# Autodesk Inventor assembly: Intake Angled
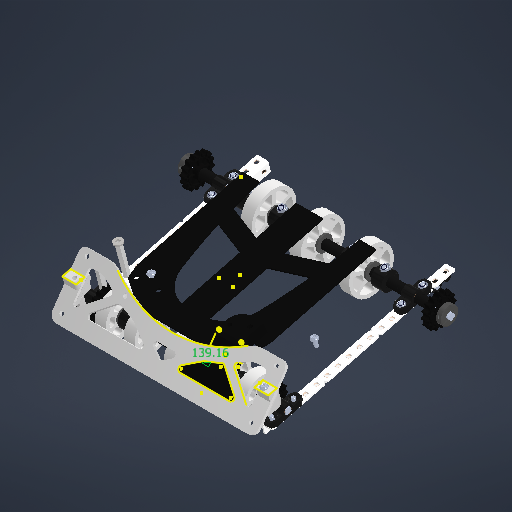
[picture p0: Inventor's stored thumbnail of the model, 512x512]
Saved by Autodesk Inventor 2025 (Build 290162000, 162)
## iProperties
Created: 2024-12-18
Part Number: Intake Angled
Document SubType Name: Assembly
Designer: Juan
Author: Juan
## Documents named in this file (38)
- C:\Users\Juan\Documents\GitHub\ATUM-VRC-High-Stakes-CAD\Robot\Subassemblies\Intake Angled.iam
- C:\Users\Juan\Documents\GitHub\ATUM-VRC-High-Stakes-CAD\VEX-CAD-Inventor\Motion\Shaft HS\Shaft HS\Shaft HS 9.0 in.ipt
- C:\Users\Juan\Documents\GitHub\ATUM-VRC-High-Stakes-CAD\VEX-CAD-Inventor\Motion\Shaft HS\Shaft HS.ipt
- C:\Users\Juan\Documents\GitHub\ATUM-VRC-High-Stakes-CAD\VEX-CAD-Inventor\Structure\Angle\Aluminum 1x1\Alu Angle 1x1x17.ipt
- C:\Users\Juan\Documents\GitHub\ATUM-VRC-High-Stakes-CAD\VEX-CAD-Inventor\Motion\Shaft HS\HS Pillow Bearing Block.ipt
- C:\Users\Juan\Documents\GitHub\ATUM-VRC-High-Stakes-CAD\VEX-CAD-Inventor\Motion\Sprockets\6P Sprocket\6P 16T Sprocket, No Insert.iam
- C:\Users\Juan\Documents\GitHub\ATUM-VRC-High-Stakes-CAD\VEX-CAD-Inventor\Motion\Sprockets\6P Sprocket.iam
- C:\Users\Juan\Documents\GitHub\ATUM-VRC-High-Stakes-CAD\VEX-CAD-Inventor\Structure\Hardware\Screw Steel - Star\SScrew Star Threaded .375.ipt
- C:\Users\Juan\Documents\GitHub\ATUM-VRC-High-Stakes-CAD\VEX-CAD-Inventor\Structure\Hardware\Screw Steel - Star.ipt
- C:\Users\Juan\Documents\GitHub\ATUM-VRC-High-Stakes-CAD\VEX-CAD-Inventor\Structure\Standoff\Standoff 1.50.ipt
- C:\Users\Juan\Documents\GitHub\ATUM-VRC-High-Stakes-CAD\VEX-CAD-Inventor\Structure\Standoff.ipt
- C:\Users\Juan\Documents\GitHub\ATUM-VRC-High-Stakes-CAD\VEX-CAD-Inventor\Motion\1-Post Bearing Flat Hex Retainer.ipt
- C:\Users\Juan\Documents\GitHub\ATUM-VRC-High-Stakes-CAD\VEX-CAD-Inventor\Motion\Shaft HS\Shaft HS\Shaft HS 12.0 in.ipt
- C:\Users\Juan\Documents\GitHub\ATUM-VRC-High-Stakes-CAD\VEX-CAD-Inventor\Motion\Shaft HS\HS Shaft Collar.ipt
- C:\Users\Juan\Documents\GitHub\ATUM-VRC-High-Stakes-CAD\VEX-CAD-Inventor\Motion\Shaft HS\HS Spacer\HSpacer .5000.ipt
- C:\Users\Juan\Documents\GitHub\ATUM-VRC-High-Stakes-CAD\VEX-CAD-Inventor\Motion\Shaft HS\HS Spacer.ipt
- C:\Users\Juan\Documents\GitHub\ATUM-VRC-High-Stakes-CAD\VEX-CAD-Inventor\Motion\Shaft HS\Low Profile HS Shaft Collar.ipt
- C:\Users\Juan\Documents\GitHub\ATUM-VRC-High-Stakes-CAD\VEX-CAD-Inventor\Motion\Shaft HS\HS Spacer\HSpacer .2500.ipt
- C:\Users\Juan\Documents\GitHub\ATUM-VRC-High-Stakes-CAD\Robot\Subassemblies\2.0 Flex Wheel with Insert.iam
- C:\Users\Juan\Documents\GitHub\ATUM-VRC-High-Stakes-CAD\VEX-CAD-Inventor\Structure\Hardware\Nut Thin Nylock.ipt
- C:\Users\Juan\Documents\GitHub\ATUM-VRC-High-Stakes-CAD\VEX-CAD-Inventor\Structure\Hardware\Screw Steel - Star\SScrew Star Smooth .625.ipt
- C:\Users\Juan\Documents\GitHub\ATUM-VRC-High-Stakes-CAD\VEX-CAD-Inventor\Motion\Shaft HS\HS Spacer\HSpacer .1250.ipt
- C:\Users\Juan\Documents\GitHub\ATUM-VRC-High-Stakes-CAD\VEX-CAD-Inventor\Motion\Shaft HS\HS Spacer\HSpacer .0625.ipt
- C:\Users\Juan\Documents\GitHub\ATUM-VRC-High-Stakes-CAD\VEX-CAD-Inventor\Structure\Hardware\Screw Steel - Star\SScrew Star Smooth .375.ipt
- C:\Users\Juan\Documents\GitHub\ATUM-VRC-High-Stakes-CAD\Robot\Subassemblies\1.625 Flex Wheel with Insert.iam
- C:\Users\Juan\Documents\GitHub\ATUM-VRC-High-Stakes-CAD\Protobot\Intake (Metal).ipt
- C:\Users\Juan\Documents\GitHub\ATUM-VRC-High-Stakes-CAD\VEX-CAD-Inventor\Motion\Spacers\Washer Steel\SWasher .375 OD x .062500.ipt
- C:\Users\Juan\Documents\GitHub\ATUM-VRC-High-Stakes-CAD\VEX-CAD-Inventor\Motion\Spacers\Washer Steel.ipt
- C:\Users\Juan\Documents\GitHub\ATUM-VRC-High-Stakes-CAD\VEX-CAD-Inventor\Motion\Spacers\Washer Steel\SWasher .375 OD x .015625.ipt
- C:\Users\Juan\Documents\GitHub\ATUM-VRC-High-Stakes-CAD\Protobot\Intake Hood.ipt
- C:\Users\Juan\Documents\GitHub\ATUM-VRC-High-Stakes-CAD\VEX-CAD-Inventor\Structure\Standoff\Standoff .75.ipt
- C:\Users\Juan\Documents\GitHub\ATUM-VRC-High-Stakes-CAD\VEX-CAD-Inventor\Motion\Spacers\Spacer Nylon .375 OD\NSpacer .375 OD x .500.ipt
- C:\Users\Juan\Documents\GitHub\ATUM-VRC-High-Stakes-CAD\VEX-CAD-Inventor\Motion\Spacers\Spacer Nylon .375 OD.ipt
- C:\Users\Juan\Documents\GitHub\ATUM-VRC-High-Stakes-CAD\Protobot\Intake Angle Mount.ipt
- C:\Users\Juan\Documents\GitHub\ATUM-VRC-High-Stakes-CAD\Protobot\Intake Angle Mount_MIR.ipt
- C:\Users\Juan\Documents\GitHub\ATUM-VRC-High-Stakes-CAD\Protobot\Intake Angle Spacer.ipt
- C:\Users\Juan\Documents\GitHub\ATUM-VRC-High-Stakes-CAD\Protobot\Intake Angle Spacer_MIR.ipt
- C:\Users\Juan\Documents\GitHub\ATUM-VRC-High-Stakes-CAD\Protobot\Intake Hood Mount.ipt
## Components (103 placed, 30 different names)
1. Shaft HS 9.0 in:1
2. Alu Angle 1x1x17:1
3. HS Pillow Bearing Block:4
4. Alu Angle 1x1x17:2 — Rigid:32, Rigid:56
5. HS Pillow Bearing Block:1 — Rigid:57
6. HS Pillow Bearing Block:2 — Rotational:1
7. 6P 16T Sprocket, No Insert:1 [sub-assembly]
8. 6P 16T Sprocket, No Insert:2 [sub-assembly]
9. SScrew Star Threaded .375:1
10. Standoff 1.50:2
11. Standoff 1.50:3
12. 1-Post Bearing Flat Hex Retainer:1
13. HS Pillow Bearing Block:3
14. Shaft HS 12.0 in:2
15. 6P 16T Sprocket, No Insert:3 [sub-assembly]
16. 6P 16T Sprocket, No Insert:4 [sub-assembly]
17. HS Shaft Collar:1
18. HS Shaft Collar:2
19. HSpacer .5000:1
20. HSpacer .5000:2
21. HSpacer .5000:3
22. HSpacer .5000:4
23. Low Profile HS Shaft Collar:1
24. Low Profile HS Shaft Collar:2
25. HS Shaft Collar:3
26. HS Shaft Collar:4
27. HSpacer .2500:5
28. HSpacer .2500:6
29. 2.0 Flex Wheel with Insert:1 [sub-assembly]
30. 1-Post Bearing Flat Hex Retainer:2
31. 2.0 Flex Wheel with Insert:2 [sub-assembly]
32. 2.0 Flex Wheel with Insert:3 [sub-assembly]
33. HSpacer .5000:7
34. Nut Thin Nylock:1
35. HSpacer .5000:8
36. SScrew Star Smooth .625:2
37. SScrew Star Smooth .625:3
38. SScrew Star Smooth .625:4
39. SScrew Star Smooth .625:5
40. Nut Thin Nylock:2
41. Nut Thin Nylock:3
42. Nut Thin Nylock:4
43. HSpacer .5000:9
44. HSpacer .5000:10
45. HSpacer .1250:11
46. HSpacer .1250:12
47. HSpacer .0625:13
48. HSpacer .1250:14
49. HSpacer .1250:15
50. HSpacer .0625:16
51. HSpacer .0625:17
52. Nut Thin Nylock:5
53. Nut Thin Nylock:6
54. Nut Thin Nylock:7
55. Nut Thin Nylock:8
56. SScrew Star Smooth .375:6
57. SScrew Star Smooth .375:7
58. SScrew Star Smooth .375:8
59. SScrew Star Smooth .375:9
60. SScrew Star Smooth .375:14
61. SScrew Star Smooth .375:15
62. SScrew Star Smooth .375:16
63. SScrew Star Smooth .375:17
64. 1.625 Flex Wheel with Insert:1 [sub-assembly]
65. 1.625 Flex Wheel with Insert:2 [sub-assembly]
66. 1.625 Flex Wheel with Insert:3 [sub-assembly]
67. 1.625 Flex Wheel with Insert:4 [sub-assembly]
68. 1.625 Flex Wheel with Insert:5 [sub-assembly]
69. HSpacer .5000:18
70. HSpacer .1250:19
71. HSpacer .1250:20
72. HSpacer .5000:21
73. HSpacer .5000:22
74. HSpacer .5000:23
75. HS Shaft Collar:5
76. Nut Thin Nylock:9
77. SScrew Star Smooth .625:18
78. HS Shaft Collar:6
79. Nut Thin Nylock:10
80. SScrew Star Smooth .625:19
81. HSpacer .1250:24
82. HSpacer .1250:25
83. Standoff 1.50:5 — Rigid:32, Rigid:36
84. SWasher .375 OD x .062500:5 — Rigid:36
85. SWasher .375 OD x .015625:6
86. Intake Hood:1 — Rigid:50, Mate:127
87. SScrew Star Smooth .375:29 — Mate:127
88. SScrew Star Smooth .375:32
89. Nut Thin Nylock:12 — Rigid:50
90. Nut Thin Nylock:17
91. SScrew Star Smooth .375:33 — Rigid:56
92. Standoff .75:7 — Rotational:1, Mate:132, Mate:133
93. Standoff .75:8 — Rigid:57, Rigid:58, Mate:130
94. Intake (Metal):1
95. NSpacer .375 OD x .500:1 — Rigid:58, Mate:128
96. Intake (Metal):2 — Flush:2, Mate:129, Flush:3, Mate:131, Mate:134, Mate:135, Mate:137, Flush:4, Mate:139, Mate:140, Mate:141
97. Intake Angle Mount:1 — Mate:128, Flush:2, Mate:129, Mate:130, Mate:136
98. Intake Angle Mount_MIR:1 — Flush:3, Mate:131, Mate:132, Mate:133, Mate:134, Mate:138
99. Intake Angle Spacer:1 — Mate:135, Mate:136, Rigid:59
100. Intake Angle Spacer_MIR:1 — Mate:137, Mate:138, Flush:4
101. SScrew Star Smooth .375:34 — Rigid:59
102. Intake Hood Mount:1 — Mate:139, Mate:140, Mate:141
103. SScrew Star Smooth .375:35
## Relationships (175: Mate 126, WeldJoint 34, CylindricalJoint 9, Flush 4, Angle 1, RevoluteJoint 1)
- [Mate]: Alu Angle 1x1x17:1 ↔ HS Pillow Bearing Block:1
- [Mate]: Alu Angle 1x1x17:1 ↔ HS Pillow Bearing Block:1
- [Mate]: Alu Angle 1x1x17:1 ↔ HS Pillow Bearing Block:1
- [Mate]: Shaft HS 9.0 in:1 ↔ HS Pillow Bearing Block:1
- [Mate]: Alu Angle 1x1x17:2 ↔ HS Pillow Bearing Block:2
- [Mate]: Alu Angle 1x1x17:2 ↔ HS Pillow Bearing Block:2
- [Mate]: Alu Angle 1x1x17:2 ↔ HS Pillow Bearing Block:2
- [Mate]: Shaft HS 9.0 in:1 ↔ HS Pillow Bearing Block:2
- [Mate]: Shaft HS 9.0 in:1 ↔ 6P 16T Sprocket, No Insert:2
- [Mate]: Shaft HS 9.0 in:1 ↔ 6P 16T Sprocket, No Insert:1
- [Mate]: Alu Angle 1x1x17:1 ↔ SScrew Star Threaded .375:1
- [Mate]: Alu Angle 1x1x17:1 ↔ 6P 16T Sprocket, No Insert:2
- [Mate]: Alu Angle 1x1x17:1 ↔ SScrew Star Threaded .375:1
- [Mate]: Alu Angle 1x1x17:1 ↔ Alu Angle 1x1x17:2
- [Mate]: HS Pillow Bearing Block:1 ↔ Standoff 1.50:2
- [Mate]: HS Pillow Bearing Block:1 ↔ Standoff 1.50:2
- [Mate]: HS Pillow Bearing Block:2 ↔ Standoff 1.50:3
- [Mate]: HS Pillow Bearing Block:2 ↔ Standoff 1.50:3
- [Mate]: Alu Angle 1x1x17:2 ↔ HS Pillow Bearing Block:3
- [Mate]: Alu Angle 1x1x17:2 ↔ HS Pillow Bearing Block:3
- [Mate]: Alu Angle 1x1x17:2 ↔ HS Pillow Bearing Block:3
- [Mate]: Shaft HS 12.0 in:2 ↔ 6P 16T Sprocket, No Insert:3
- [Mate]: Shaft HS 12.0 in:2 ↔ 6P 16T Sprocket, No Insert:4
- [Mate]: Shaft HS 12.0 in:2 ↔ 2.0 Flex Wheel with Insert:3
- [Mate]: Shaft HS 12.0 in:2 ↔ 2.0 Flex Wheel with Insert:2
- [Mate]: Shaft HS 12.0 in:2 ↔ 2.0 Flex Wheel with Insert:1
- [Mate]: Shaft HS 12.0 in:2 ↔ HSpacer .5000:4
- [Mate]: Shaft HS 12.0 in:2 ↔ HSpacer .5000:4
- [Mate]: Shaft HS 12.0 in:2 ↔ HS Shaft Collar:1
- [Mate]: Shaft HS 12.0 in:2 ↔ HS Shaft Collar:1
- [Mate]: Shaft HS 12.0 in:2 ↔ HSpacer .5000:1
- [Mate]: Shaft HS 12.0 in:2 ↔ HSpacer .5000:1
- [Mate]: HSpacer .5000:1 ↔ HSpacer .5000:4
- [Mate]: HS Shaft Collar:1 ↔ HSpacer .5000:4
- [Mate]: HS Shaft Collar:1 ↔ 2.0 Flex Wheel with Insert:3
- [Mate]: HSpacer .5000:1 ↔ 2.0 Flex Wheel with Insert:2
- [Mate]: Shaft HS 12.0 in:2 ↔ HS Shaft Collar:2
- [Mate]: Shaft HS 12.0 in:2 ↔ HS Shaft Collar:2
- [Mate]: Shaft HS 12.0 in:2 ↔ HSpacer .5000:3
- [Mate]: Shaft HS 12.0 in:2 ↔ HSpacer .5000:3
- [Mate]: Shaft HS 12.0 in:2 ↔ HSpacer .5000:2
- [Mate]: Shaft HS 12.0 in:2 ↔ HSpacer .5000:2
- [Mate]: HSpacer .5000:2 ↔ 2.0 Flex Wheel with Insert:2
- [Mate]: HSpacer .5000:2 ↔ HSpacer .5000:3
- [Mate]: HS Shaft Collar:2 ↔ HSpacer .5000:3
- [Mate]: HS Shaft Collar:2 ↔ 2.0 Flex Wheel with Insert:1
- [Mate] (36.1696 mm): Alu Angle 1x1x17:1 ↔ 2.0 Flex Wheel with Insert:3
- [Mate]: Shaft HS 12.0 in:2 ↔ Low Profile HS Shaft Collar:2
- [Mate]: Shaft HS 12.0 in:2 ↔ Low Profile HS Shaft Collar:2
- [Mate]: 6P 16T Sprocket, No Insert:3 ↔ Low Profile HS Shaft Collar:2
- [Mate]: Shaft HS 12.0 in:2 ↔ Low Profile HS Shaft Collar:1
- [Mate]: Shaft HS 12.0 in:2 ↔ Low Profile HS Shaft Collar:1
- [Mate]: 6P 16T Sprocket, No Insert:4 ↔ Low Profile HS Shaft Collar:1
- [Mate]: Shaft HS 12.0 in:2 ↔ HS Shaft Collar:3
- [Mate]: Shaft HS 12.0 in:2 ↔ HS Shaft Collar:3
- [Mate]: Shaft HS 12.0 in:2 ↔ HS Shaft Collar:4
- [Mate]: Shaft HS 12.0 in:2 ↔ HS Shaft Collar:4
- [Mate]: Shaft HS 12.0 in:2 ↔ HSpacer .2500:5
- [Mate]: Shaft HS 12.0 in:2 ↔ HSpacer .2500:5
- [Mate]: Shaft HS 12.0 in:2 ↔ HSpacer .2500:6
- [Mate]: Shaft HS 12.0 in:2 ↔ HSpacer .2500:6
- [Mate]: HSpacer .2500:6 ↔ 2.0 Flex Wheel with Insert:3
- [Mate]: HSpacer .2500:5 ↔ 2.0 Flex Wheel with Insert:1
- [Mate]: HS Shaft Collar:4 ↔ HSpacer .2500:5
- [Mate]: HS Shaft Collar:3 ↔ HSpacer .2500:6
- [WeldJoint]: HS Shaft Collar:3 ↔ SScrew Star Smooth .625:2
- [WeldJoint]: HS Shaft Collar:1 ↔ SScrew Star Smooth .625:5
- [WeldJoint]: HS Shaft Collar:2 ↔ SScrew Star Smooth .625:4
- [WeldJoint]: HS Shaft Collar:4 ↔ SScrew Star Smooth .625:3
- [WeldJoint]: HS Shaft Collar:3 ↔ Nut Thin Nylock:1
- [WeldJoint]: HS Shaft Collar:4 ↔ Nut Thin Nylock:2
- [WeldJoint]: HS Shaft Collar:2 ↔ Nut Thin Nylock:3
- [WeldJoint]: HS Shaft Collar:1 ↔ Nut Thin Nylock:4
- [WeldJoint]: HS Shaft Collar:3 ↔ HSpacer .5000:7
- [WeldJoint]: HS Shaft Collar:4 ↔ HSpacer .5000:9
- [Mate]: Shaft HS 12.0 in:2 ↔ HSpacer .5000:8
- [Mate]: 6P 16T Sprocket, No Insert:3 ↔ HSpacer .5000:8
- [Mate]: Shaft HS 12.0 in:2 ↔ HSpacer .5000:10
- [Mate]: 6P 16T Sprocket, No Insert:4 ↔ HSpacer .5000:10
- [Mate]: Shaft HS 12.0 in:2 ↔ HSpacer .1250:12
- [Mate]: HSpacer .5000:10 ↔ HSpacer .1250:12
- [Mate]: HSpacer .5000:9 ↔ HSpacer .1250:11
- [Mate]: HSpacer .5000:9 ↔ HSpacer .1250:11
- [Mate]: HSpacer .1250:11 ↔ HSpacer .0625:13
- [Mate]: HSpacer .1250:11 ↔ HSpacer .0625:13
- [Mate]: HSpacer .5000:8 ↔ HSpacer .1250:14
- [Mate]: HSpacer .5000:8 ↔ HSpacer .1250:14
- [Mate]: HSpacer .1250:14 ↔ HSpacer .0625:16
- [Mate]: HSpacer .1250:14 ↔ HSpacer .0625:16
- [Mate]: HSpacer .5000:7 ↔ HSpacer .1250:15
- [Mate]: HSpacer .5000:7 ↔ HSpacer .1250:15
- [Mate]: HSpacer .1250:15 ↔ HSpacer .0625:17
- [Mate]: HSpacer .1250:15 ↔ HSpacer .0625:17
- [WeldJoint]: HS Pillow Bearing Block:3 ↔ Nut Thin Nylock:7
- [WeldJoint]: HS Pillow Bearing Block:3 ↔ Nut Thin Nylock:8
- [WeldJoint]: Alu Angle 1x1x17:1 ↔ SScrew Star Smooth .375:6
- [WeldJoint]: Alu Angle 1x1x17:1 ↔ SScrew Star Smooth .375:7
- [WeldJoint]: Alu Angle 1x1x17:2 ↔ SScrew Star Smooth .375:9
- [WeldJoint]: Alu Angle 1x1x17:2 ↔ SScrew Star Smooth .375:8
- [WeldJoint]: Alu Angle 1x1x17:2 ↔ SScrew Star Smooth .375:15
- [WeldJoint]: Alu Angle 1x1x17:2 ↔ SScrew Star Smooth .375:14
- [WeldJoint]: Alu Angle 1x1x17:1 ↔ SScrew Star Smooth .375:17
- [WeldJoint]: Alu Angle 1x1x17:1 ↔ SScrew Star Smooth .375:16
- [CylindricalJoint]: Shaft HS 9.0 in:1 ↔ 1.625 Flex Wheel with Insert:1
- [CylindricalJoint]: Shaft HS 9.0 in:1 ↔ 1.625 Flex Wheel with Insert:5
- [Mate]: 1.625 Flex Wheel with Insert:5 ↔ HSpacer .5000:18
- [Mate]: 1.625 Flex Wheel with Insert:5 ↔ HSpacer .1250:19
- [Mate]: 1.625 Flex Wheel with Insert:5 ↔ HSpacer .1250:19
- [Mate]: HSpacer .5000:18 ↔ HSpacer .1250:19
- [Mate]: 1.625 Flex Wheel with Insert:5 ↔ HSpacer .1250:20
- [Mate]: 1.625 Flex Wheel with Insert:5 ↔ HSpacer .1250:20
- [Mate]: 1.625 Flex Wheel with Insert:5 ↔ HSpacer .5000:21
- [Mate]: HSpacer .1250:20 ↔ HSpacer .5000:21
- [Mate]: 1.625 Flex Wheel with Insert:5 ↔ HSpacer .5000:23
- [Mate]: HSpacer .5000:18 ↔ HSpacer .5000:23
- [Mate]: 1.625 Flex Wheel with Insert:5 ↔ HSpacer .5000:22
- [Mate]: HSpacer .5000:21 ↔ HSpacer .5000:22
- [Mate]: 1.625 Flex Wheel with Insert:1 ↔ HSpacer .5000:23
- [CylindricalJoint]: Shaft HS 9.0 in:1 ↔ 1.625 Flex Wheel with Insert:4
- [Mate]: 1.625 Flex Wheel with Insert:4 ↔ HSpacer .5000:22
- [CylindricalJoint]: Shaft HS 9.0 in:1 ↔ 1.625 Flex Wheel with Insert:3
- [CylindricalJoint]: Shaft HS 9.0 in:1 ↔ 1.625 Flex Wheel with Insert:2
- [WeldJoint]: HS Shaft Collar:5 ↔ SScrew Star Smooth .625:18
- [WeldJoint]: HS Shaft Collar:5 ↔ Nut Thin Nylock:9
- [WeldJoint]: HS Shaft Collar:6 ↔ SScrew Star Smooth .625:19
- [WeldJoint]: HS Shaft Collar:6 ↔ Nut Thin Nylock:10
- [CylindricalJoint]: Shaft HS 9.0 in:1 ↔ HS Shaft Collar:5
- [CylindricalJoint]: Shaft HS 9.0 in:1 ↔ HS Shaft Collar:6
- [Mate]: 6P 16T Sprocket, No Insert:1 ↔ 1.625 Flex Wheel with Insert:2
- [Mate]: 1.625 Flex Wheel with Insert:2 ↔ HS Shaft Collar:6
- [Mate]: 6P 16T Sprocket, No Insert:2 ↔ 1.625 Flex Wheel with Insert:3
- [Mate]: 1.625 Flex Wheel with Insert:3 ↔ HS Shaft Collar:5
- [Mate]: Alu Angle 1x1x17:2 ↔ 6P 16T Sprocket, No Insert:1
- [Flush]: HS Shaft Collar:5 ↔ HS Shaft Collar:6
- [Angle] (0 deg): Shaft HS 9.0 in:1 ↔ HS Shaft Collar:5
- [CylindricalJoint]: Shaft HS 9.0 in:1 ↔ HSpacer .1250:25
- [Mate]: HS Shaft Collar:5 ↔ HSpacer .1250:25
- [Mate]: 1.625 Flex Wheel with Insert:1 ↔ HSpacer .1250:25
- [CylindricalJoint]: Shaft HS 9.0 in:1 ↔ HSpacer .1250:24
- [Mate]: 1.625 Flex Wheel with Insert:4 ↔ HSpacer .1250:24
- [Mate]: Alu Angle 1x1x17:1 ↔ HS Pillow Bearing Block:4
- [Mate]: Alu Angle 1x1x17:1 ↔ HS Pillow Bearing Block:4
- [Mate]: Alu Angle 1x1x17:1 ↔ HS Pillow Bearing Block:4
- [Mate]: HS Pillow Bearing Block:4 ↔ Shaft HS 12.0 in:2
- [WeldJoint]: HS Pillow Bearing Block:4 ↔ Nut Thin Nylock:6
- [WeldJoint]: HS Pillow Bearing Block:4 ↔ Nut Thin Nylock:5
- [Mate]: Alu Angle 1x1x17:1 ↔ 1-Post Bearing Flat Hex Retainer:2
- [Mate]: SScrew Star Threaded .375:1 ↔ 1-Post Bearing Flat Hex Retainer:2
- Rigid:32 [WeldJoint]: Alu Angle 1x1x17:2 ↔ Standoff 1.50:5
- [WeldJoint]: SWasher .375 OD x .062500:5 ↔ SWasher .375 OD x .015625:6
- Rigid:36 [WeldJoint]: Standoff 1.50:5 ↔ SWasher .375 OD x .062500:5
- Rigid:50 [WeldJoint]: Intake Hood:1 ↔ Nut Thin Nylock:12
- Rigid:56 [WeldJoint]: Alu Angle 1x1x17:2 ↔ SScrew Star Smooth .375:33
- Mate:127: Intake Hood:1 ↔ SScrew Star Smooth .375:29
- Rigid:57 [WeldJoint]: HS Pillow Bearing Block:1 ↔ Standoff .75:8
- Rotational:1 [RevoluteJoint]: HS Pillow Bearing Block:2 ↔ Standoff .75:7
- Rigid:58 [WeldJoint]: Standoff .75:8 ↔ NSpacer .375 OD x .500:1
- Mate:128: NSpacer .375 OD x .500:1 ↔ Intake Angle Mount:1
- Flush:2: Intake (Metal):2 ↔ Intake Angle Mount:1
- Mate:129: Intake (Metal):2 ↔ Intake Angle Mount:1
- Mate:130: Standoff .75:8 ↔ Intake Angle Mount:1
- Flush:3: Intake (Metal):2 ↔ Intake Angle Mount_MIR:1
- Mate:131: Intake (Metal):2 ↔ Intake Angle Mount_MIR:1
- Mate:132: Standoff .75:7 ↔ Intake Angle Mount_MIR:1
- Mate:133: Standoff .75:7 ↔ Intake Angle Mount_MIR:1
- Mate:134: Intake (Metal):2 ↔ Intake Angle Mount_MIR:1
- Mate:135: Intake (Metal):2 ↔ Intake Angle Spacer:1
- Mate:136: Intake Angle Mount:1 ↔ Intake Angle Spacer:1
- Mate:137: Intake (Metal):2 ↔ Intake Angle Spacer_MIR:1
- Mate:138: Intake Angle Mount_MIR:1 ↔ Intake Angle Spacer_MIR:1
- Flush:4: Intake (Metal):2 ↔ Intake Angle Spacer_MIR:1
- Rigid:59 [WeldJoint]: Intake Angle Spacer:1 ↔ SScrew Star Smooth .375:34
- Mate:139: Intake (Metal):2 ↔ Intake Hood Mount:1
- Mate:140: Intake (Metal):2 ↔ Intake Hood Mount:1
- Mate:141: Intake (Metal):2 ↔ Intake Hood Mount:1
## Named parameters: d2183_d2114 = 0 mm, d2184_d2118 = 0 mm, d2185_d2183_d2114 = 0 mm, d2186_d2184_d2118 = 0 mm, d178_d177 = 0 mm
